# Autodesk Inventor assembly: Ensamble
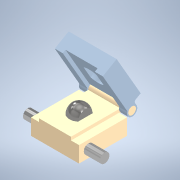
[picture p0: Inventor's stored thumbnail of the model, 180x180]
Saved by Autodesk Inventor 2021 (Build 250183000, 183)
## iProperties
Created: 2021-03-19
Part Number: Ensamble
Document SubType Name: Assembly
Designer: trejo
Author: trejo
## Documents named in this file (5)
- C:\Users\trejo\Documents\Octavo Cuatrimestre\3D Design\homework\Actividad 5\Rocker Box\Ensamble.iam
- C:\Users\trejo\Documents\Octavo Cuatrimestre\3D Design\homework\Actividad 5\Rocker Box\Rocker Box Base.0001.ipt
- C:\Users\trejo\Documents\Octavo Cuatrimestre\3D Design\homework\Actividad 5\Rocker Box\Rocker Box Cylinder.0001.ipt
- C:\Users\trejo\Documents\Octavo Cuatrimestre\3D Design\homework\Actividad 5\Rocker Box\Rocker Box Ball.0001.ipt
- C:\Users\trejo\Documents\Octavo Cuatrimestre\3D Design\homework\Actividad 5\Rocker Box\Rocker Box Top.0001.ipt
## Components (4 placed, 4 different names)
1. Rocker Box Base.0001:1 — Slider:1, Rotational:1, Cylindrical:1
2. Rocker Box Cylinder.0001:1 — Slider:1
3. Rocker Box Ball.0001:1 — Rotational:1
4. Rocker Box Top.0001:1 — Cylindrical:1
## Relationships (3: TranslationJoint 1, RevoluteJoint 1, CylindricalJoint 1)
- Slider:1 [TranslationJoint] (20 mm): Rocker Box Base.0001:1 ↔ Rocker Box Cylinder.0001:1
- Rotational:1 [RevoluteJoint]: Rocker Box Base.0001:1 ↔ Rocker Box Ball.0001:1
- Cylindrical:1: Rocker Box Base.0001:1 ↔ Rocker Box Top.0001:1
